# Autodesk Inventor assembly: 305-03
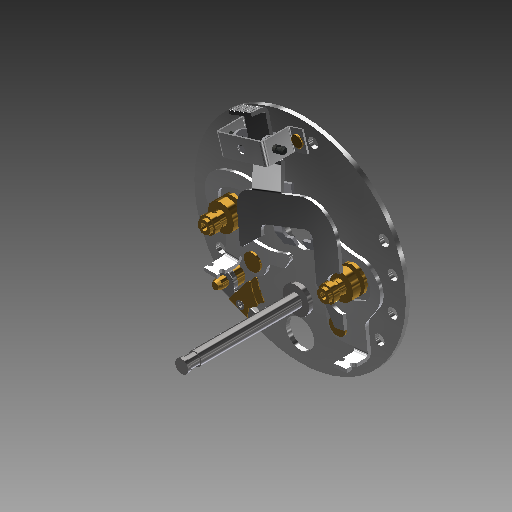
[picture p0: Inventor's stored thumbnail of the model, 512x512]
Saved by Autodesk Inventor 2019 (Build 230136000, 136)
## iProperties
Company: Autodesk Inc.
Created: 2012-01-26
Part Number: 305-03
Document SubType Name: Assembly
Designer: Autodesk Inc.
Mass: 26.4522 g
Surface Area: 148.815 cm^2
Volume: 7.5295 cm^3
Density: 3.51314 g/cm^3
Author: Inventor
## Documents named in this file (17)
- C:\TEMP\Fishing Rod\Workspaces\Winding Assembly.iam
- C:\TEMP\Fishing Rod\Workspaces\Winding Assembly Plate.ipt
- C:\TEMP\Fishing Rod\Workspaces\Winding Assembly Base Ring.ipt
- C:\TEMP\Fishing Rod\Workspaces\Drag Lock Guide.ipt
- C:\TEMP\Fishing Rod\Workspaces\Drag Lock Pivot Pin.ipt
- C:\TEMP\Fishing Rod\Workspaces\Drag Lock.ipt
- C:\TEMP\Fishing Rod\Workspaces\Crankshaft Spindle.ipt
- C:\TEMP\Fishing Rod\Workspaces\Swing Arm - Left.ipt
- C:\TEMP\Fishing Rod\Workspaces\Swing Arm - Right.ipt
- C:\TEMP\Fishing Rod\Workspaces\Swing Arm Pivot Pin.ipt
- C:\TEMP\Fishing Rod\Workspaces\Pivot Pin.ipt
- C:\TEMP\Fishing Rod\Workspaces\Drag Lever Guide Bracket.ipt
- C:\TEMP\Fishing Rod\Workspaces\Drag Lever Spring Arm.ipt
- C:\TEMP\Fishing Rod\Workspaces\Drag Lever Spring Pin.ipt
- C:\TEMP\Fishing Rod\Workspaces\Drag Lever.ipt
- C:\TEMP\Fishing Rod\Libraries\Content Center Files\en-US\Rivet GOST 12639-80\Rivet A 1.4x2 GOST 12639-80.ipt
- C:\TEMP\Fishing Rod\Workspaces\Rivet.ipt
## Components (19 placed, 16 different names)
1. Winding Assembly Plate:1 — Insert:1, Mate:1, Insert:2, Insert:5, Insert:6, Insert:7, Insert:8, Insert:9, Insert:10, Insert:11, Insert:12, Mate:3
2. Winding Assembly Base Ring:1 — Insert:1, Mate:1
3. Drag Lock Guide:1 — Insert:4, Angle:1, Insert:15
4. Drag Lock Pivot Pin:1 — Insert:2, Insert:3
5. Drag Lock:1 — Insert:3, Insert:4, Angle:1
6. Crankshaft Spindle:1 — Insert:5
7. Swing Arm - Left:1 — Insert:8
8. Swing Arm - Right:1 — Insert:6
9. Swing Arm Pivot Pin:1 — Insert:7
10. Swing Arm Pivot Pin:2 — Insert:9
11. Pivot Pin:1 — Insert:10
12. Pivot Pin:2 — Insert:11
13. Drag Lever Guide Bracket:1 — Insert:12, Insert:16, Insert:18, Mate:3, Insert:19
14. Drag Lever Spring Arm:1 — Insert:14, Mate:2
15. Drag Lever Spring Pin:1 — Insert:14, Insert:18
16. Drag Lever:1 — Mate:2
17. Rivet GOST 12639-80 A 1.4x2:1 — Insert:15
18. Rivet:1 — Insert:16
19. Rivet:2 — Insert:19
## Relationships (21: Insert 17, Mate 3, Angle 1)
- Insert:1: Winding Assembly Plate:1 ↔ Winding Assembly Base Ring:1
- Mate:1: Winding Assembly Plate:1 ↔ Winding Assembly Base Ring:1
- Insert:2: Winding Assembly Plate:1 ↔ Drag Lock Pivot Pin:1
- Insert:3: Drag Lock Pivot Pin:1 ↔ Drag Lock:1
- Insert:4: Drag Lock Guide:1 ↔ Drag Lock:1
- Angle:1 (0 deg): Drag Lock Guide:1 ↔ Drag Lock:1
- Insert:5: Winding Assembly Plate:1 ↔ Crankshaft Spindle:1
- Insert:6: Winding Assembly Plate:1 ↔ Swing Arm - Right:1
- Insert:7: Winding Assembly Plate:1 ↔ Swing Arm Pivot Pin:1
- Insert:8: Winding Assembly Plate:1 ↔ Swing Arm - Left:1
- Insert:9: Winding Assembly Plate:1 ↔ Swing Arm Pivot Pin:2
- Insert:10: Winding Assembly Plate:1 ↔ Pivot Pin:1
- Insert:11: Winding Assembly Plate:1 ↔ Pivot Pin:2
- Insert:12: Winding Assembly Plate:1 ↔ Drag Lever Guide Bracket:1
- Insert:14: Drag Lever Spring Arm:1 ↔ Drag Lever Spring Pin:1
- Insert:15: Drag Lock Guide:1 ↔ Rivet GOST 12639-80 A 1.4x2:1
- Insert:16: Drag Lever Guide Bracket:1 ↔ Rivet:1
- Insert:18: Drag Lever Guide Bracket:1 ↔ Drag Lever Spring Pin:1
- Mate:2: Drag Lever Spring Arm:1 ↔ Drag Lever:1
- Mate:3: Winding Assembly Plate:1 ↔ Drag Lever Guide Bracket:1
- Insert:19: Drag Lever Guide Bracket:1 ↔ Rivet:2
